# Autodesk Inventor assembly: drivetrain
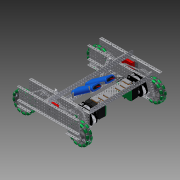
[picture p0: Inventor's stored thumbnail of the model, 180x180]
Saved by Autodesk Inventor 2014 SP1 (Build 180222100, 222)
## iProperties
Created: 2013-10-19
Part Number: drivetrain
Document SubType Name: Assembly
Designer: RyanHughes
Author: RyanHughes
## Documents named in this file (7)
- C:\Users\Ryan\Desktop\sw\toss up 2ed A bot\drivetrain\drivetrain.iam
- C:\Users\Ryan\Desktop\sw\toss up 2ed A bot\drivetrain\one side of drive.iam
- C:\Users\Ryan\Desktop\sw\lib\Aperture VEX CAD Library\Metal\L Bar\2 x 25 - A bot 2 drive connector.ipt
- C:\Users\Ryan\Desktop\sw\lib\Aperture VEX CAD Library\Metal\Plate\5 x 14.ipt
- C:\Users\Ryan\Desktop\sw\lib\Aperture VEX CAD Library\Motors\motor controller\29.iam
- C:\Users\Ryan\Desktop\sw\toss up 2ed A bot\drivetrain\cross support\cross support.iam
- C:\Users\Ryan\Desktop\sw\toss up 2ed A bot\drivetrain\one side of drive_MIR.iam
## Components (11 placed, 6 different names)
1. 2 x 25 - A bot 2 drive connector:1 — Mate:2, Flush:3, Flush:4, Mate:14, Mate:15, Mate:16, Flush:5, Flush:6, Mate:18, Flush:9, Flush:10
2. 5 x 14:1 — Mate:2, Flush:3, Flush:4, Mate:3, Mate:4, Mate:5, Mate:6, Mate:7, Mate:8, Mate:9, Mate:10
3. cross support:1 [sub-assembly] — Mate:13, Mate:17, Flush:7, Flush:8
4. one side of drive:1 [sub-assembly] — Mate:16, Flush:5, Flush:6, Mate:17, Flush:7, Flush:8
5. one side of drive_MIR:1 [sub-assembly] — Mate:18, Flush:9, Flush:10
6. 29:1 [sub-assembly] — Mate:3, Mate:4, Mate:5, Mate:6
7. 29:6 [sub-assembly]
8. 29:2 [sub-assembly] — Mate:7, Mate:8, Mate:9, Mate:10
9. 29:3 [sub-assembly]
10. 29:4 [sub-assembly]
11. 29:5 [sub-assembly]
## Component patterns: (2 elements), (2 elements, first: 29:1), (2 elements, first: 29:2), Component Pattern 1:2 (2 elements)
## Relationships (23: Mate 15, Flush 8)
- Mate:2: 2 x 25 - A bot 2 drive connector:1 ↔ 5 x 14:1
- Flush:3: 2 x 25 - A bot 2 drive connector:1 ↔ 5 x 14:1
- Flush:4: 2 x 25 - A bot 2 drive connector:1 ↔ 5 x 14:1
- Mate:3: 5 x 14:1 ↔ 29:1
- Mate:4 (2.3114 mm): 5 x 14:1 ↔ 29:1
- Mate:5 (2.3114 mm): 5 x 14:1 ↔ 29:1
- Mate:6 (2.3114 mm): 5 x 14:1 ↔ 29:1
- Mate:7: 5 x 14:1 ↔ 29:2
- Mate:8 (2.3114 mm): 5 x 14:1 ↔ 29:2
- Mate:9 (2.3114 mm): 5 x 14:1 ↔ 29:2
- Mate:10 (2.3114 mm): 5 x 14:1 ↔ 29:2
- Mate:13 (-12.7 mm): cross support:1
- Mate:14: 2 x 25 - A bot 2 drive connector:1
- Mate:15: 2 x 25 - A bot 2 drive connector:1
- Mate:16: 2 x 25 - A bot 2 drive connector:1 ↔ one side of drive:1
- Flush:5: 2 x 25 - A bot 2 drive connector:1 ↔ one side of drive:1
- Flush:6: 2 x 25 - A bot 2 drive connector:1 ↔ one side of drive:1
- Mate:17: cross support:1 ↔ one side of drive:1
- Flush:7: cross support:1 ↔ one side of drive:1
- Flush:8: cross support:1 ↔ one side of drive:1
- Mate:18: 2 x 25 - A bot 2 drive connector:1 ↔ one side of drive_MIR:1
- Flush:9: 2 x 25 - A bot 2 drive connector:1 ↔ one side of drive_MIR:1
- Flush:10: 2 x 25 - A bot 2 drive connector:1 ↔ one side of drive_MIR:1
## Named parameters: q = 2.3114 mm
